# Autodesk Inventor assembly: POM_T5_04
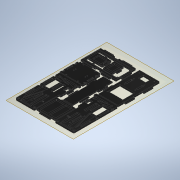
[picture p0: Inventor's stored thumbnail of the model, 180x180]
Saved by Autodesk Inventor 2020 (Build 240168000, 168)
## iProperties
Created: 2021-08-27
Part Number: POM_T5_04
Document SubType Name: Assembly
Designer: Masato
Author: Masato
## Documents named in this file (11)
- C:\Users\naoki\Documents\Inventor\CitBrains\git_clone\OpenPlatform4_0\コックピットCAM\OpenPlatform_ver3_0\cam\POM_T5_04.iam
- C:\Users\naoki\Documents\Inventor\CitBrains\git_clone\OpenPlatform4_0\コックピットCAM\OpenPlatform_ver3_0\cam\Disposable_Board.ipt
- C:\Users\naoki\Documents\Inventor\CitBrains\git_clone\OpenPlatform4_0\コックピットCAM\OpenPlatform_ver3_0\UpperBody\Cockpit\Cockpit_lower_back_door.ipt
- C:\Users\naoki\Documents\Inventor\CitBrains\git_clone\OpenPlatform4_0\コックピットCAM\OpenPlatform_ver3_0\UpperBody\Cockpit\Cockpit_lower_bottom_frame.ipt
- C:\Users\naoki\Documents\Inventor\CitBrains\git_clone\OpenPlatform4_0\コックピットCAM\OpenPlatform_ver3_0\UpperBody\Cockpit\Cockpit_lower_front_frame.ipt
- C:\Users\naoki\Documents\Inventor\CitBrains\git_clone\OpenPlatform4_0\コックピットCAM\OpenPlatform_ver3_0\UpperBody\Cockpit\Cockpit_upper_bottom_frame.ipt
- C:\Users\naoki\Documents\Inventor\CitBrains\git_clone\OpenPlatform4_0\コックピットCAM\OpenPlatform_ver3_0\UpperBody\Cockpit\Cockpit_upper_front_frame.ipt
- C:\Users\naoki\Documents\Inventor\CitBrains\git_clone\OpenPlatform4_0\コックピットCAM\OpenPlatform_ver3_0\UpperBody\Cockpit\Cockpit_upper_middle_frame.ipt
- C:\Users\naoki\Documents\Inventor\CitBrains\git_clone\OpenPlatform4_0\コックピットCAM\OpenPlatform_ver3_0\UpperBody\Cockpit\Cockpit_upper_side_frame.ipt
- C:\Users\naoki\Documents\Inventor\CitBrains\git_clone\OpenPlatform4_0\コックピットCAM\OpenPlatform_ver3_0\UpperBody\Cockpit\Cockpit_upper_side_frame_MIR.ipt
- C:\Users\naoki\Documents\Inventor\CitBrains\git_clone\OpenPlatform4_0\コックピットCAM\OpenPlatform_ver3_0\UpperBody\Cockpit\Cockpit_upper_top_frame.ipt
## Components (10 placed, 10 different names)
1. Disposable_Board:1 — メイト:2, メイト:1, フラッシュ:1, フラッシュ:2, フラッシュ:3, フラッシュ:9, フラッシュ:10
2. Cockpit_lower_back_door:1 — メイト:12, 正接:1, メイト:23, メイト:24
3. Cockpit_lower_bottom_frame:1 — メイト:8, メイト:16, メイト:17
4. Cockpit_lower_front_frame:1 — メイト:11, メイト:22, メイト:24
5. Cockpit_upper_bottom_frame:1 — メイト:10, メイト:19, メイト:25
6. Cockpit_upper_front_frame:1 — メイト:9, フラッシュ:7, フラッシュ:8, メイト:14, メイト:15, メイト:17
7. Cockpit_upper_middle_frame:1 — メイト:13, フラッシュ:6, メイト:21, メイト:22, 正接:1, メイト:23, メイト:25
8. Cockpit_upper_side_frame:1 — メイト:4, フラッシュ:3, フラッシュ:7, メイト:14, メイト:16, フラッシュ:9, メイト:18
9. Cockpit_upper_side_frame_MIR:1 — メイト:6, フラッシュ:8, メイト:15, メイト:19
10. Cockpit_upper_top_frame:1 — メイト:5, フラッシュ:6, フラッシュ:10, メイト:18, メイト:21
## Relationships (31: Mate 22, Flush 8, Tangent 1)
- メイト:2 [Mate]: Disposable_Board:1
- メイト:1 [Mate]: Disposable_Board:1
- フラッシュ:1 [Flush]: Disposable_Board:1
- フラッシュ:2 [Flush]: Disposable_Board:1
- メイト:4 [Mate]: Cockpit_upper_side_frame:1
- メイト:5 [Mate]: Cockpit_upper_top_frame:1
- メイト:6 [Mate]: Cockpit_upper_side_frame_MIR:1
- メイト:8 [Mate]: Cockpit_lower_bottom_frame:1
- メイト:9 [Mate]: Cockpit_upper_front_frame:1
- メイト:10 [Mate]: Cockpit_upper_bottom_frame:1
- メイト:11 [Mate]: Cockpit_lower_front_frame:1
- メイト:12 [Mate]: Cockpit_lower_back_door:1
- メイト:13 [Mate]: Cockpit_upper_middle_frame:1
- フラッシュ:3 [Flush] (2 mm): Disposable_Board:1 ↔ Cockpit_upper_side_frame:1
- フラッシュ:6 [Flush]: Cockpit_upper_middle_frame:1 ↔ Cockpit_upper_top_frame:1
- フラッシュ:7 [Flush]: Cockpit_upper_front_frame:1 ↔ Cockpit_upper_side_frame:1
- フラッシュ:8 [Flush]: Cockpit_upper_front_frame:1 ↔ Cockpit_upper_side_frame_MIR:1
- メイト:14 [Mate] (2.5 mm): Cockpit_upper_front_frame:1 ↔ Cockpit_upper_side_frame:1
- メイト:15 [Mate] (2.5 mm): Cockpit_upper_front_frame:1 ↔ Cockpit_upper_side_frame_MIR:1
- メイト:16 [Mate] (3.5 mm): Cockpit_lower_bottom_frame:1 ↔ Cockpit_upper_side_frame:1
- メイト:17 [Mate] (2.5 mm): Cockpit_lower_bottom_frame:1 ↔ Cockpit_upper_front_frame:1
- フラッシュ:9 [Flush] (4 mm): Disposable_Board:1 ↔ Cockpit_upper_side_frame:1
- フラッシュ:10 [Flush] (2 mm): Disposable_Board:1 ↔ Cockpit_upper_top_frame:1
- メイト:18 [Mate] (2.5 mm): Cockpit_upper_side_frame:1 ↔ Cockpit_upper_top_frame:1
- メイト:19 [Mate] (2.5 mm): Cockpit_upper_bottom_frame:1 ↔ Cockpit_upper_side_frame_MIR:1
- メイト:21 [Mate] (2.5 mm): Cockpit_upper_middle_frame:1 ↔ Cockpit_upper_top_frame:1
- メイト:22 [Mate] (2.5 mm): Cockpit_lower_front_frame:1 ↔ Cockpit_upper_middle_frame:1
- 正接:1 [Tangent] (2.5 mm): Cockpit_lower_back_door:1 ↔ Cockpit_upper_middle_frame:1
- メイト:23 [Mate] (2.5 mm): Cockpit_lower_back_door:1 ↔ Cockpit_upper_middle_frame:1
- メイト:24 [Mate] (2.5 mm): Cockpit_lower_back_door:1 ↔ Cockpit_lower_front_frame:1
- メイト:25 [Mate] (2.5 mm): Cockpit_upper_bottom_frame:1 ↔ Cockpit_upper_middle_frame:1
